# Autodesk Inventor assembly: EBF_910.1-eb-flow
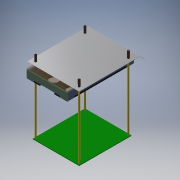
[picture p0: Inventor's stored thumbnail of the model, 180x180]
Saved by Autodesk Inventor 2019 (Build 230136000, 136)
## iProperties
Created: 2019-03-05
Part Number: EBF_910.1-eb-flow
Document SubType Name: Assembly
Designer: Rene
Author: Rene
## Documents named in this file (5)
- C:\dev\c-scape\hardponics\dwg\eb_flow\EBF_910.1-eb-flow.iam
- C:\dev\c-scape\hardponics\dwg\eb_flow\XGEN_hotbed-pcb.ipt
- C:\dev\c-scape\hardponics\dwg\eb_flow\EBF_900.1-water-tray_with_cups.iam
- C:\dev\c-scape\hardponics\dwg\eb_flow\XGEN_simsun-pcb.ipt
- C:\dev\c-scape\hardponics\dwg\eb_flow\XGEN_spacer-long.ipt
## Components (7 placed, 4 different names)
1. XGEN_hotbed-pcb:1 — Mate:1, Mate:2, Mate:3, Mate:4, Mate:5
2. EBF_900.1-water-tray_with_cups:1 [sub-assembly] — Mate:1, Mate:2
3. XGEN_simsun-pcb:1 — Mate:3, Mate:4, Mate:5, Mate:6, Mate:7, Mate:8, Mate:9, Mate:10, Mate:11, Mate:12, Mate:13
4. XGEN_spacer-long:1 — Mate:8, Mate:9
5. XGEN_spacer-long:2 — Mate:6, Mate:7
6. XGEN_spacer-long:3 — Mate:12, Mate:13
7. XGEN_spacer-long:4 — Mate:10, Mate:11
## Relationships (13: Mate 13)
- Mate:1: XGEN_hotbed-pcb:1 ↔ EBF_900.1-water-tray_with_cups:1
- Mate:2: XGEN_hotbed-pcb:1 ↔ EBF_900.1-water-tray_with_cups:1
- Mate:3: XGEN_hotbed-pcb:1 ↔ XGEN_simsun-pcb:1
- Mate:4: XGEN_hotbed-pcb:1 ↔ XGEN_simsun-pcb:1
- Mate:5 (230 mm): XGEN_hotbed-pcb:1 ↔ XGEN_simsun-pcb:1
- Mate:6: XGEN_simsun-pcb:1 ↔ XGEN_spacer-long:2
- Mate:7: XGEN_simsun-pcb:1 ↔ XGEN_spacer-long:2
- Mate:8: XGEN_simsun-pcb:1 ↔ XGEN_spacer-long:1
- Mate:9: XGEN_simsun-pcb:1 ↔ XGEN_spacer-long:1
- Mate:10: XGEN_simsun-pcb:1 ↔ XGEN_spacer-long:4
- Mate:11: XGEN_simsun-pcb:1 ↔ XGEN_spacer-long:4
- Mate:12: XGEN_simsun-pcb:1 ↔ XGEN_spacer-long:3
- Mate:13: XGEN_simsun-pcb:1 ↔ XGEN_spacer-long:3
